# Autodesk Inventor assembly: Heat_shield
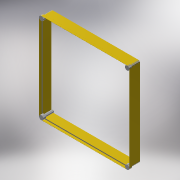
[picture p0: Inventor's stored thumbnail of the model, 180x180]
Saved by Autodesk Inventor 2020 (Build 240168000, 168)
## iProperties
Created: 2018-05-08
Part Number: Heat_shield
Document SubType Name: Assembly
Designer: PC  USER
Author: PC  USER
## Documents named in this file (3)
- C:\Users\pc-konvi\Documents\Lobola\open_source_scrabble\CAD model\heat shield\Heat_shield.iam
- C:\Users\pc-konvi\Documents\Lobola\open_source_scrabble\CAD model\heat shield\thin nuts.ipt
- C:\Users\pc-konvi\Documents\Lobola\open_source_scrabble\CAD model\heat shield\foil_shield.ipt
## Components (8 placed, 2 different names)
1. thin nuts:1 — Flush:3, Mate:7, Flush:4, Flush:5, Mate:14
2. thin nuts:2 — Flush:2, Flush:3, Mate:9, Flush:6, Mate:16
3. thin nuts:3 — Flush:1, Flush:2, Mate:6, Flush:4, Mate:13
4. thin nuts:4 — Flush:1, Mate:8, Flush:5, Flush:6, Mate:15
5. foil_shield:1 — Mate:6, Angle:1, Mate:10, Mate:12, Mate:13, Mate:18, Mate:20
6. foil_shield:2 — Mate:7, Angle:2, Mate:10, Mate:11, Mate:14, Mate:17, Mate:21
7. foil_shield:3 — Mate:8, Angle:3, Mate:11, Mate:15, Mate:18, Mate:19
8. foil_shield:4 — Mate:9, Mate:12, Mate:16, Mate:17, Mate:19, Mate:22
## Relationships (26: Mate 17, Flush 6, Angle 3)
- Flush:1: thin nuts:3 ↔ thin nuts:4
- Flush:2: thin nuts:2 ↔ thin nuts:3
- Flush:3: thin nuts:1 ↔ thin nuts:2
- Mate:6: thin nuts:3 ↔ foil_shield:1
- Mate:7: thin nuts:1 ↔ foil_shield:2
- Mate:8: thin nuts:4 ↔ foil_shield:3
- Mate:9: thin nuts:2 ↔ foil_shield:4
- Angle:1 (0 deg): foil_shield:1
- Angle:2 (0 deg): foil_shield:2
- Angle:3 (180 deg): foil_shield:3
- Flush:4: thin nuts:1 ↔ thin nuts:3
- Flush:5: thin nuts:1 ↔ thin nuts:4
- Flush:6: thin nuts:2 ↔ thin nuts:4
- Mate:10: foil_shield:1 ↔ foil_shield:2
- Mate:11: foil_shield:2 ↔ foil_shield:3
- Mate:12: foil_shield:1 ↔ foil_shield:4
- Mate:13: thin nuts:3 ↔ foil_shield:1
- Mate:14: thin nuts:1 ↔ foil_shield:2
- Mate:15: thin nuts:4 ↔ foil_shield:3
- Mate:16: thin nuts:2 ↔ foil_shield:4
- Mate:17 (200 mm): foil_shield:2 ↔ foil_shield:4
- Mate:18 (200 mm): foil_shield:1 ↔ foil_shield:3
- Mate:19: foil_shield:3 ↔ foil_shield:4
- Mate:20 (100 mm): foil_shield:1
- Mate:21 (100 mm): foil_shield:2
- Mate:22: foil_shield:4
